# Autodesk Inventor assembly: hubble_telescope_assembly
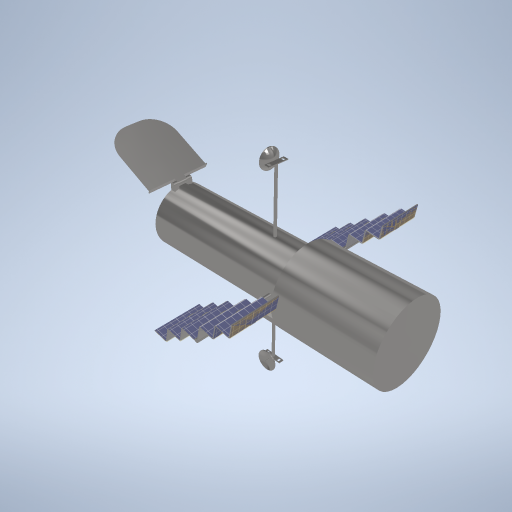
[picture p0: Inventor's stored thumbnail of the model, 512x512]
Saved by Autodesk Inventor 2024 (Build 280153000, 153)
## iProperties
Created: 2024-04-14
Part Number: hubble_telescope_assembly
Document SubType Name: Assembly
Designer: soham
Author: soham
## Documents named in this file (7)
- \\Mac\Home\Documents\Soham-UoA\Documents\CAD - 115\hubble_telescope_assembly.iam
- \\Mac\Home\Documents\Soham-UoA\Documents\CAD - 115\hubble_main_body.ipt
- \\Mac\Home\Documents\Soham-UoA\Documents\CAD - 115\hubble_solar_panel.ipt
- \\Mac\Home\Documents\Soham-UoA\Documents\CAD - 115\hubble_solar_panel_MIR.ipt
- \\Mac\Home\Documents\Soham-UoA\Documents\CAD - 115\aperature_panel.ipt
- \\Mac\Home\Documents\Soham-UoA\Documents\CAD - 115\hubble_antenna.ipt
- \\Mac\Home\Documents\Soham-UoA\Documents\CAD - 115\hubble_antenna_MIR.ipt
## Components (6 placed, 6 different names)
1. hubble_main_body:1 — Rotational:1, Rotational:2, Rotational:3, Rotational:4, Rotational:5
2. hubble_solar_panel:1 — Rotational:1, Rotation:1
3. hubble_solar_panel_MIR:1 — Rotational:2, Rotation:1
4. aperature_panel:1 — Rotational:3
5. hubble_antenna:1 — Rotational:4
6. hubble_antenna_MIR:1 — Rotational:5
## Relationships (6: RevoluteJoint 5, RelateRotation 1)
- Rotational:1 [RevoluteJoint]: hubble_main_body:1 ↔ hubble_solar_panel:1
- Rotational:2 [RevoluteJoint]: hubble_main_body:1 ↔ hubble_solar_panel_MIR:1
- Rotation:1 [RelateRotation] (1 ul): hubble_solar_panel:1 ↔ hubble_solar_panel_MIR:1
- Rotational:3 [RevoluteJoint]: hubble_main_body:1 ↔ aperature_panel:1
- Rotational:4 [RevoluteJoint]: hubble_main_body:1 ↔ hubble_antenna:1
- Rotational:5 [RevoluteJoint]: hubble_main_body:1 ↔ hubble_antenna_MIR:1
## Named parameters: Finish1_Area = 4574.81
note: some values were not read from the file. Shown as the stored number, unit unknown: "Finish1_Area".
